# Autodesk Inventor assembly: Trapezoid Polycarbonate End Ramp Assembly
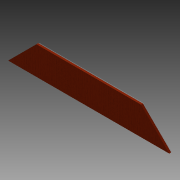
[picture p0: Inventor's stored thumbnail of the model, 180x180]
Saved by Autodesk Inventor 2015 (Build 190159000, 159)
## iProperties
Created: 2015-01-21
Part Number: Trapezoid Polycarbonate End Ramp Assembly
Document SubType Name: Assembly
Designer: peters
Author: peters
## Documents named in this file (3)
- C:\Users\peters\Documents\FIRST-Team-1719-CAD-Team\2015 Playing Field\Team 1719 Practice Field\Scoring Platform Version 2 - Construction Design\Ramp - End - Trapezoid Assembly.iam
- C:\Users\peters\Documents\FIRST-Team-1719-CAD-Team\2015 Playing Field\Team 1719 Practice Field\Scoring Platform Version 2 - Construction Design\Ramp - End - Trapezoid Plywood 375.ipt
- C:\Users\peters\Documents\FIRST-Team-1719-CAD-Team\2015 Playing Field\Team 1719 Practice Field\Scoring Platform Version 2 - Construction Design\Ramp - End - Trapezoid Polycarbonate 125.ipt
## Components (2 placed, 2 different names)
1. Ramp - End - Trapezoid Plywood 375:1 — Mate:1, Flush:1, Flush:2
2. Ramp - End - Trapezoid Polycarbonate 125:1 — Mate:1, Flush:1, Flush:2
## Relationships (3: Flush 2, Mate 1)
- Mate:1: Ramp - End - Trapezoid Plywood 375:1 ↔ Ramp - End - Trapezoid Polycarbonate 125:1
- Flush:1: Ramp - End - Trapezoid Plywood 375:1 ↔ Ramp - End - Trapezoid Polycarbonate 125:1
- Flush:2: Ramp - End - Trapezoid Plywood 375:1 ↔ Ramp - End - Trapezoid Polycarbonate 125:1
